# Autodesk Inventor assembly: Montiert
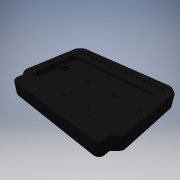
[picture p0: Inventor's stored thumbnail of the model, 180x180]
Saved by Autodesk Inventor 2017 SP1 (Build 210196100, 196)
## iProperties
Part Number: Montiert
Material: Generisch
Document SubType Name: Assembly
Designer: aXe
Author: aXe
## Documents named in this file (4)
- C:\Users\aXe\Dropbox\Elektronik\aXe_Dashboard240XL\Gehäuse\Montiert.iam
- C:\Users\aXe\Dropbox\Elektronik\aXe_Dashboard240XL\Gehäuse\GehäuseDeckel.ipt
- C:\Users\aXe\Dropbox\Elektronik\aXe_Dashboard240XL\Gehäuse\Platine\PCB_SingleLedRow.iam
- C:\Users\aXe\Dropbox\Elektronik\aXe_Dashboard240XL\Gehäuse\Boden_v2.ipt
## Components (3 placed, 3 different names)
1. GehäuseDeckel:1 — Fluchtend:1, Passend:1, Passend:2, Fluchtend:2, Fluchtend:3, Fluchtend:5
2. PCB_SingleLedRow:1 [sub-assembly] — Fluchtend:1, Passend:1, Passend:2, Fluchtend:6
3. Boden_v2:1 — Fluchtend:3, Fluchtend:5, Fluchtend:6
## Relationships (7: Flush 5, Mate 2)
- Fluchtend:1 [Flush]: GehäuseDeckel:1 ↔ PCB_SingleLedRow:1
- Passend:1 [Mate] (0.1 mm): GehäuseDeckel:1 ↔ PCB_SingleLedRow:1
- Passend:2 [Mate] (3.05 mm): GehäuseDeckel:1 ↔ PCB_SingleLedRow:1
- Fluchtend:2 [Flush] (0.2 mm): GehäuseDeckel:1
- Fluchtend:3 [Flush]: GehäuseDeckel:1 ↔ Boden_v2:1
- Fluchtend:5 [Flush]: GehäuseDeckel:1 ↔ Boden_v2:1
- Fluchtend:6 [Flush]: PCB_SingleLedRow:1 ↔ Boden_v2:1
